# Autodesk Inventor assembly: Ensamble - 1
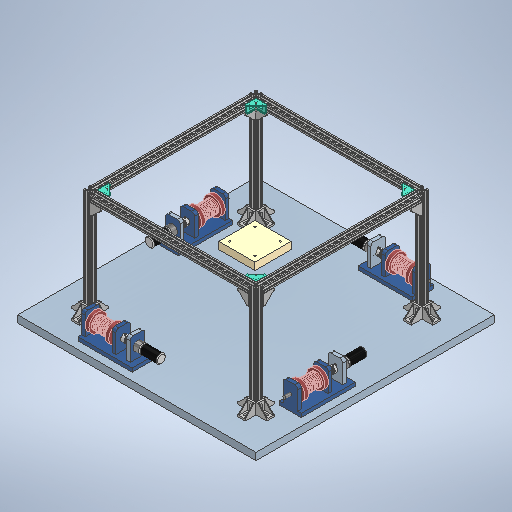
[picture p0: Inventor's stored thumbnail of the model, 512x512]
Saved by Autodesk Inventor 2026 (Build 300175050, 175E)
## iProperties
Created: 2025-06-30
Part Number: Ensamble - 1
Document SubType Name: Assembly
Designer: piero
Author: piero
## Documents named in this file (9)
- C:\Users\piero\OneDrive\Documentos\UTEC\Ciclo 2025-1\PFC_1\ModeloBase\CAD\Ensamble - 1.iam
- C:\Users\piero\OneDrive\Documentos\UTEC\Ciclo 2025-1\PFC_1\ModeloBase\CAD\Mesa.ipt
- C:\Users\piero\OneDrive\Documentos\UTEC\Ciclo 2025-1\PFC_1\ModeloBase\CAD\V-slot.ipt
- C:\Users\piero\OneDrive\Documentos\UTEC\Ciclo 2025-1\PFC_1\ModeloBase\CAD\Ensamblaje2.iam
- C:\Users\piero\OneDrive\Documentos\UTEC\Ciclo 2025-1\PFC_1\ModeloBase\CAD\Plataforma.ipt
- C:\Users\piero\OneDrive\Documentos\UTEC\Ciclo 2025-1\PFC_1\ModeloBase\CAD\Esquinero.ipt
- C:\Users\piero\OneDrive\Documentos\UTEC\Ciclo 2025-1\PFC_1\ModeloBase\CAD\V-slot_2.ipt
- C:\Users\piero\OneDrive\Documentos\UTEC\Ciclo 2025-1\PFC_1\ModeloBase\CAD\Soporte gancho.ipt
- C:\Users\piero\OneDrive\Documentos\UTEC\Ciclo 2025-1\PFC_1\ModeloBase\CAD\Gancho.ipt
## Components (46 placed, 8 different names)
1. Mesa:1 — Coincidencia:10, Coincidencia:15, Coincidencia:16, Ángulo:1, Coincidencia:17, Ángulo:2, Coincidencia:22, Coincidencia:26
2. V-slot:1 — Coincidencia:3, Nivelación:5, Nivelación:6, Nivelación:7, Nivelación:8, Coincidencia:4, Coincidencia:11, Nivelación:13, Nivelación:14, Coincidencia:14, Ángulo:3, Ángulo:4, Coincidencia:25, Nivelación:15, Nivelación:16
3. V-slot:2 — Nivelación:9, Nivelación:10, Coincidencia:5, Coincidencia:6, Nivelación:11, Nivelación:12
4. V-slot:3 — Coincidencia:7, Coincidencia:8, Coincidencia:9
5. V-slot:4 — Nivelación:1, Nivelación:2, Coincidencia:1, Nivelación:3, Nivelación:4, Coincidencia:2, Coincidencia:10
6. Plataforma:1
7. V-slot_2:1 — Nivelación:7, Nivelación:8, Coincidencia:4, Nivelación:9, Nivelación:10, Coincidencia:5, Coincidencia:13, Coincidencia:19, Coincidencia:28
8. V-slot_2:2 — Nivelación:1, Nivelación:2, Coincidencia:1, Coincidencia:8, Coincidencia:9
9. V-slot_2:3 — Coincidencia:6, Nivelación:11, Nivelación:12, Coincidencia:7
10. V-slot_2:4 — Nivelación:3, Nivelación:4, Coincidencia:2, Coincidencia:3, Nivelación:5, Nivelación:6, Coincidencia:12, Coincidencia:18, Coincidencia:27
11. Esquinero:6 — Coincidencia:13, Nivelación:14, Coincidencia:14
12. Esquinero:5 — Coincidencia:11, Nivelación:13, Coincidencia:12
13. Ensamblaje2:1 [sub-assembly] — Coincidencia:22
14. Soporte gancho:1 — Nivelación:16, Coincidencia:27, Coincidencia:28, Coincidencia:29
15. Gancho:1 — Coincidencia:29
16. Esquinero:11
17. Esquinero:12
18. Ensamblaje2:2 [sub-assembly]
19. Soporte gancho:2
20. Gancho:2
21. Esquinero:17
22. Esquinero:18
23. Ensamblaje2:3 [sub-assembly]
24. Soporte gancho:3
25. Gancho:3
26. Esquinero:23
27. Esquinero:24
28. Ensamblaje2:4 [sub-assembly]
29. Soporte gancho:4
30. Gancho:4
31. Esquinero:7 — Coincidencia:25, Nivelación:15, Coincidencia:26
32. Esquinero:8
33. Esquinero:9
34. Esquinero:10
35. Esquinero:13
36. Esquinero:14
37. Esquinero:15
38. Esquinero:16
39. Esquinero:19
40. Esquinero:20
41. Esquinero:21
42. Esquinero:22
43. Esquinero:25
44. Esquinero:26
45. Esquinero:27
46. Esquinero:28
## Component patterns: (4 elements, first: Esquinero:6 + Esquinero:5 + Ensamblaje2:1 + Soporte gancho:1 + Gancho:1), (4 elements, first: Esquinero:7), Patrón de componentes 2:2 (4 elements), Patrón de componentes 2:3 (4 elements), Patrón de componentes 2:4 (4 elements)
## Relationships (49: Mate 29, Flush 16, Angle 4)
- Nivelación:1 [Flush]: V-slot:4 ↔ V-slot_2:2
- Nivelación:2 [Flush]: V-slot:4 ↔ V-slot_2:2
- Coincidencia:1 [Mate]: V-slot:4 ↔ V-slot_2:2
- Nivelación:3 [Flush]: V-slot:4 ↔ V-slot_2:4
- Nivelación:4 [Flush]: V-slot:4 ↔ V-slot_2:4
- Coincidencia:2 [Mate]: V-slot:4 ↔ V-slot_2:4
- Coincidencia:3 [Mate]: V-slot:1 ↔ V-slot_2:4
- Nivelación:5 [Flush]: V-slot:1 ↔ V-slot_2:4
- Nivelación:6 [Flush]: V-slot:1 ↔ V-slot_2:4
- Nivelación:7 [Flush]: V-slot:1 ↔ V-slot_2:1
- Nivelación:8 [Flush]: V-slot:1 ↔ V-slot_2:1
- Coincidencia:4 [Mate]: V-slot:1 ↔ V-slot_2:1
- Nivelación:9 [Flush]: V-slot:2 ↔ V-slot_2:1
- Nivelación:10 [Flush]: V-slot:2 ↔ V-slot_2:1
- Coincidencia:5 [Mate]: V-slot:2 ↔ V-slot_2:1
- Coincidencia:6 [Mate]: V-slot:2 ↔ V-slot_2:3
- Nivelación:11 [Flush]: V-slot:2 ↔ V-slot_2:3
- Nivelación:12 [Flush]: V-slot:2 ↔ V-slot_2:3
- Coincidencia:7 [Mate]: V-slot:3 ↔ V-slot_2:3
- Coincidencia:8 [Mate]: V-slot:3 ↔ V-slot_2:2
- Coincidencia:9 [Mate]: V-slot:3 ↔ V-slot_2:2
- Coincidencia:10 [Mate]: Mesa:1 ↔ V-slot:4
- Coincidencia:11 [Mate]: V-slot:1 ↔ Esquinero:5
- Nivelación:13 [Flush]: V-slot:1 ↔ Esquinero:5
- Coincidencia:12 [Mate]: V-slot_2:4 ↔ Esquinero:5
- Coincidencia:13 [Mate]: V-slot_2:1 ↔ Esquinero:6
- Nivelación:14 [Flush]: V-slot:1 ↔ Esquinero:6
- Coincidencia:14 [Mate]: V-slot:1 ↔ Esquinero:6
- Coincidencia:15 [Mate]: Mesa:1
- Coincidencia:16 [Mate]: Mesa:1
- Ángulo:1 [Angle] (0 deg): Mesa:1
- Coincidencia:17 [Mate]: Mesa:1
- Ángulo:2 [Angle] (0 deg): Mesa:1
- Coincidencia:18 [Mate]: V-slot_2:4
- Ángulo:3 [Angle] (0 deg): V-slot:1
- Coincidencia:19 [Mate]: V-slot_2:1
- Ángulo:4 [Angle] (0 deg): V-slot:1
- Coincidencia:20 [Mate]
- Coincidencia:21 [Mate]
- Coincidencia:22 [Mate]: Mesa:1 ↔ Ensamblaje2:1
- Coincidencia:23 [Mate]
- Coincidencia:24 [Mate]
- Coincidencia:25 [Mate]: V-slot:1 ↔ Esquinero:7
- Nivelación:15 [Flush]: V-slot:1 ↔ Esquinero:7
- Coincidencia:26 [Mate]: Mesa:1 ↔ Esquinero:7
- Nivelación:16 [Flush]: V-slot:1 ↔ Soporte gancho:1
- Coincidencia:27 [Mate]: V-slot_2:4 ↔ Soporte gancho:1
- Coincidencia:28 [Mate]: V-slot_2:1 ↔ Soporte gancho:1
- Coincidencia:29 [Mate]: Soporte gancho:1 ↔ Gancho:1
